# Autodesk Inventor assembly: Intake assembly
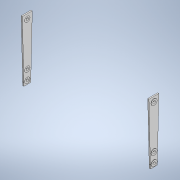
[picture p0: Inventor's stored thumbnail of the model, 180x180]
Saved by Autodesk Inventor 2020 (Build 240168000, 168)
## iProperties
Created: 2020-02-06
Part Number: Intake assembly
Document SubType Name: Assembly
Designer: aidan
Author: aidan
## Documents named in this file (3)
- C:\Users\aidan\Desktop\T3 Robotics\CAD\Intake assembly.iam
- C:\Users\aidan\Desktop\T3 Robotics\CAD\Intake - Side Panel.ipt
- C:\Users\aidan\Desktop\T3 Robotics\CAD\Bearing for THUNDER.ipt
## Components (8 placed, 2 different names)
1. Intake - Side Panel:1 — Mate:1, Insert:1, Insert:2, Insert:3
2. Intake - Side Panel:2 — Mate:1, Insert:4, Insert:5, Insert:6
3. Bearing for THUNDER:1 — Insert:1
4. Bearing for THUNDER:2 — Insert:6
5. Bearing for THUNDER:3 — Insert:5
6. Bearing for THUNDER:4 — Insert:4
7. Bearing for THUNDER:5 — Insert:3
8. Bearing for THUNDER:6 — Insert:2
## Relationships (7: Insert 6, Mate 1)
- Mate:1 (647.7 mm): Intake - Side Panel:1 ↔ Intake - Side Panel:2
- Insert:1: Intake - Side Panel:1 ↔ Bearing for THUNDER:1
- Insert:2: Intake - Side Panel:1 ↔ Bearing for THUNDER:6
- Insert:3: Intake - Side Panel:1 ↔ Bearing for THUNDER:5
- Insert:4: Intake - Side Panel:2 ↔ Bearing for THUNDER:4
- Insert:5: Intake - Side Panel:2 ↔ Bearing for THUNDER:3
- Insert:6: Intake - Side Panel:2 ↔ Bearing for THUNDER:2
